# Autodesk Inventor assembly: pulley_small_pair
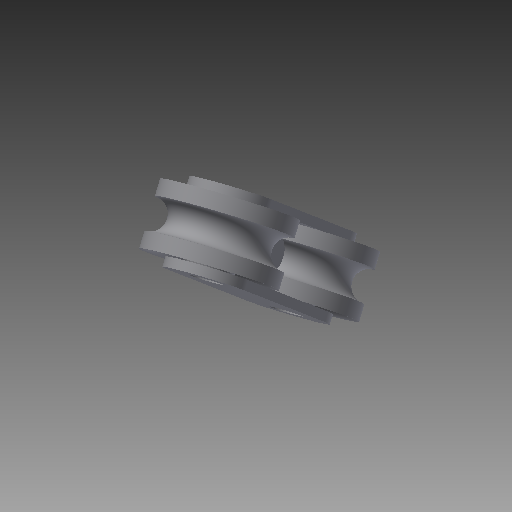
[picture p0: Inventor's stored thumbnail of the model, 512x512]
Saved by Autodesk Inventor 2019 (Build 230136000, 136)
## iProperties
Created: 2019-01-06
Part Number: pulley_small_pair
Document SubType Name: Assembly
Designer: MJ
Author: MJ
## Documents named in this file (5)
- C:\Users\MJ\Documents\AiFit-Inventor\pulley_small_pair.iam
- C:\Users\MJ\Documents\AiFit-Inventor\pulley_small.ipt
- C:\Users\MJ\Documents\AiFit-Inventor\joint.ipt
- C:\Users\MJ\Documents\AiFit-Inventor\joint_MIR.ipt
- C:\Users\MJ\Documents\AiFit-Inventor\pipe.ipt
## Components (5 placed, 4 different names)
1. pulley_small:1 — Mate:6, Rotational:2, Rotational:3
2. pulley_small:2 — Mate:5, Mate:6, Rotational:4, Rotational:5
3. joint:1 — Mate:5, Rotational:2, Rotational:4, Flush:1, Mate:7, Flush:2
4. joint_MIR:1 — Rotational:3, Rotational:5
5. pipe:1 — Flush:1, Mate:7, Flush:2
## Relationships (10: Mate 4, RevoluteJoint 4, Flush 2)
- [Mate]: pulley_small:1 ↔ pulley_small:2
- Mate:5: pulley_small:2 ↔ joint:1
- Mate:6: pulley_small:1 ↔ pulley_small:2
- Rotational:2 [RevoluteJoint]: pulley_small:1 ↔ joint:1
- Rotational:3 [RevoluteJoint]: pulley_small:1 ↔ joint_MIR:1
- Rotational:4 [RevoluteJoint]: pulley_small:2 ↔ joint:1
- Rotational:5 [RevoluteJoint]: pulley_small:2 ↔ joint_MIR:1
- Flush:1: joint:1 ↔ pipe:1
- Mate:7: joint:1 ↔ pipe:1
- Flush:2: joint:1 ↔ pipe:1
